# Autodesk Inventor assembly: main assembly
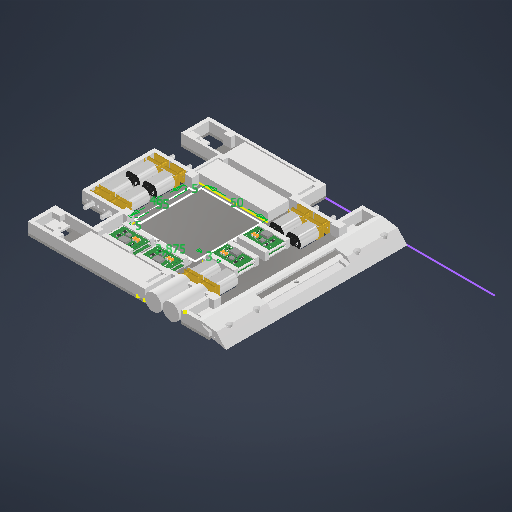
[picture p0: Inventor's stored thumbnail of the model, 512x512]
Saved by Autodesk Inventor 2026.2 (Build 302298010, 298A)
## iProperties
Created: 2026-04-27
Part Number: main assembly
Document SubType Name: Assembly
Designer: karol
Author: karol
## Documents named in this file (21)
- C:\Users\karol\OneDrive\Dokumenty\GitHub\bolt\bolt\cad\assembly\main assembly.iam
- C:\Users\karol\OneDrive\Dokumenty\GitHub\bolt\bolt\cad\ready parts\base.ipt
- C:\Users\karol\OneDrive\Dokumenty\GitHub\bolt\bolt\cad\ready parts\lewasciana.ipt
- C:\Users\karol\OneDrive\Dokumenty\GitHub\bolt\bolt\cad\ready parts\prawasciana.ipt
- C:\Users\karol\OneDrive\Dokumenty\GitHub\bolt\bolt\cad\ready parts\rmwall.ipt
- C:\Users\karol\OneDrive\Dokumenty\GitHub\bolt\bolt\cad\ready parts\lmwall.ipt
- C:\Users\karol\OneDrive\Dokumenty\GitHub\bolt\bolt\cad\ready parts\Pololu #2218 Micro Metal Gearmotor HP.ipt
- C:\Users\karol\OneDrive\Dokumenty\GitHub\bolt\bolt\cad\assembly\backmotors.iam
- C:\Users\karol\OneDrive\Dokumenty\GitHub\bolt\bolt\cad\ready parts\lewascianakoło.ipt
- C:\Users\karol\OneDrive\Dokumenty\GitHub\bolt\bolt\cad\ready parts\prawascianakolo.ipt
- C:\Users\karol\OneDrive\Dokumenty\GitHub\bolt\bolt\cad\ready parts\lfmw.ipt
- C:\Users\karol\OneDrive\Dokumenty\GitHub\bolt\bolt\cad\ready parts\rfmw.ipt
- C:\Users\karol\OneDrive\Dokumenty\GitHub\bolt\bolt\cad\ready parts\lipo.ipt
- C:\Users\karol\OneDrive\Dokumenty\GitHub\bolt\bolt\cad\assembly\plugassmbly.iam
- C:\Users\karol\OneDrive\Dokumenty\GitHub\bolt\bolt\cad\assembly\drvassembly.iam
- C:\Users\karol\OneDrive\Dokumenty\GitHub\bolt\bolt\cad\printing parts\rim-v1.ipt
- C:\Users\karol\OneDrive\Dokumenty\GitHub\bolt\bolt\cad\assembly\drvassemblylf.iam
- drvassemblylf.iam
- C:\Users\karol\OneDrive\Dokumenty\GitHub\bolt\bolt\cad\assembly\drvassemblyrf.iam
- drvassemblyrf.iam
- C:\Users\karol\OneDrive\Dokumenty\GitHub\bolt\bolt\cad\ready parts\zawiasv2.ipt
## Components (25 placed, 18 different names)
1. base:1 — Mate:1, Mate:2, Mate:3, Mate:4, Mate:5, Mate:7, Mate:15, Mate:16, Mate:17, Mate:18, Mate:21, Mate:22, Mate:23, Mate:24, Mate:28, Mate:29, Mate:30, Mate:32, Mate:33, Mate:34, Mate:35, Mate:36, Mate:37, Mate:38, Mate:39, Mate:40, Mate:41, Mate:45, Mate:47, Mate:48, Mate:68, Mate:73, Mate:74, Mate:75, Mate:80, Mate:81, Mate:82, Mate:83
2. lewasciana:1 — Mate:1, Mate:2, Mate:46, Mate:54, Mate:55, Mate:70, Mate:71, Mate:72
3. prawasciana:1 — Mate:3, Mate:4, Mate:49, Mate:56
4. rmwall:1 — Mate:5, Mate:48, Mate:49, Mate:50, Mate:51, Mate:79
5. lmwall:1 — Mate:7, Mate:52, Mate:53, Mate:54, Mate:55, Flush:1, Flush:2, Mate:61, Mate:76
6. Pololu #2218 Micro Metal Gearmotor HP:3 — Mate:17, Mate:18
7. Pololu #2218 Micro Metal Gearmotor HP:4 — Mate:15, Mate:16
8. Pololu #2218 Micro Metal Gearmotor HP:7 — Mate:21, Mate:22
9. Pololu #2218 Micro Metal Gearmotor HP:8 — Mate:23, Mate:24, Mate:60, Angle:1
10. lewascianakoło:1 — Mate:32, Mate:33, Mate:69
11. prawascianakolo:1 — Mate:28, Mate:29, Mate:30, Mate:42, Mate:43
12. backmotors:1 [sub-assembly] — Mate:34, Mate:35
13. lfmw:1 — Mate:36, Mate:37, Mate:38, Mate:52, Mate:53, Mate:77
14. rfmw:1 — Mate:39, Mate:40, Mate:41, Mate:50, Mate:51, Mate:78
15. lipo:2 — Mate:46, Mate:47
16. lipo:3 — Mate:42, Mate:43
17. lipo:4 — Mate:45, Mate:56
18. plugassmbly:1 [sub-assembly] — Mate:84, Mate:85, Mate:86, Mate:87
19. drvassembly:1 [sub-assembly] — Mate:68, Mate:69, Mate:70
20. drvassembly:2 [sub-assembly] — Mate:71, Mate:72, Mate:73
21. rim-v1:1 — Flush:1, Flush:2
22. rim-v1:2 — Mate:60, Angle:1, Mate:61
23. drvassemblylf:1 [sub-assembly] — Mate:75, Mate:78, Mate:79
24. drvassemblyrf:3 [sub-assembly] — Mate:74, Mate:76, Mate:77
25. zawiasv2:1 — Mate:80, Mate:81, Mate:82, Mate:83, Mate:84, Mate:85, Mate:86, Mate:87
## Relationships (66: Mate 63, Flush 2, Angle 1)
- Mate:1: base:1 ↔ lewasciana:1
- Mate:2: base:1 ↔ lewasciana:1
- Mate:3: base:1 ↔ prawasciana:1
- Mate:4: base:1 ↔ prawasciana:1
- Mate:5: base:1 ↔ rmwall:1
- Mate:7: base:1 ↔ lmwall:1
- Mate:15: base:1 ↔ Pololu #2218 Micro Metal Gearmotor HP:4
- Mate:16: base:1 ↔ Pololu #2218 Micro Metal Gearmotor HP:4
- Mate:17: base:1 ↔ Pololu #2218 Micro Metal Gearmotor HP:3
- Mate:18: base:1 ↔ Pololu #2218 Micro Metal Gearmotor HP:3
- Mate:21: base:1 ↔ Pololu #2218 Micro Metal Gearmotor HP:7
- Mate:22: base:1 ↔ Pololu #2218 Micro Metal Gearmotor HP:7
- Mate:23: base:1 ↔ Pololu #2218 Micro Metal Gearmotor HP:8
- Mate:24: base:1 ↔ Pololu #2218 Micro Metal Gearmotor HP:8
- Mate:28: base:1 ↔ prawascianakolo:1
- Mate:29: base:1 ↔ prawascianakolo:1
- Mate:30: base:1 ↔ prawascianakolo:1
- Mate:32: base:1 ↔ lewascianakoło:1
- Mate:33: base:1 ↔ lewascianakoło:1
- Mate:34: base:1 ↔ backmotors:1
- Mate:35: base:1 ↔ backmotors:1
- Mate:36: base:1 ↔ lfmw:1
- Mate:37: base:1 ↔ lfmw:1
- Mate:38: base:1 ↔ lfmw:1
- Mate:39: base:1 ↔ rfmw:1
- Mate:40: base:1 ↔ rfmw:1
- Mate:41: base:1 ↔ rfmw:1
- Mate:42: prawascianakolo:1 ↔ lipo:3
- Mate:43: prawascianakolo:1 ↔ lipo:3
- Mate:45: base:1 ↔ lipo:4
- Mate:46: lewasciana:1 ↔ lipo:2
- Mate:47: base:1 ↔ lipo:2
- Mate:48: base:1 ↔ rmwall:1
- Mate:49: prawasciana:1 ↔ rmwall:1
- Mate:50: rmwall:1 ↔ rfmw:1
- Mate:51: rmwall:1 ↔ rfmw:1
- Mate:52: lmwall:1 ↔ lfmw:1
- Mate:53: lmwall:1 ↔ lfmw:1
- Mate:54: lewasciana:1 ↔ lmwall:1
- Mate:55: lewasciana:1 ↔ lmwall:1
- Mate:56: prawasciana:1 ↔ lipo:4
- Flush:1: lmwall:1 ↔ rim-v1:1
- Flush:2 (0.5 mm): lmwall:1 ↔ rim-v1:1
- Mate:60: Pololu #2218 Micro Metal Gearmotor HP:8 ↔ rim-v1:2
- Angle:1 (180 deg): Pololu #2218 Micro Metal Gearmotor HP:8 ↔ rim-v1:2
- Mate:61: lmwall:1 ↔ rim-v1:2
- Mate:68: base:1 ↔ drvassembly:1
- Mate:69 (5 mm): lewascianakoło:1 ↔ drvassembly:1
- Mate:70 (20 mm): lewasciana:1 ↔ drvassembly:1
- Mate:71 (4 mm): lewasciana:1 ↔ drvassembly:2
- Mate:72 (20 mm): lewasciana:1 ↔ drvassembly:2
- Mate:73: base:1 ↔ drvassembly:2
- Mate:74: base:1 ↔ drvassemblyrf:3
- Mate:75: base:1 ↔ drvassemblylf:1
- Mate:76 (27 mm): lmwall:1 ↔ drvassemblyrf:3
- Mate:77 (8 mm): lfmw:1 ↔ drvassemblyrf:3
- Mate:78 (8 mm): rfmw:1 ↔ drvassemblylf:1
- Mate:79 (27 mm): rmwall:1 ↔ drvassemblylf:1
- Mate:80: base:1 ↔ zawiasv2:1
- Mate:81: base:1 ↔ zawiasv2:1
- Mate:82: base:1 ↔ zawiasv2:1
- Mate:83: base:1 ↔ zawiasv2:1
- Mate:84: plugassmbly:1 ↔ zawiasv2:1
- Mate:85: plugassmbly:1 ↔ zawiasv2:1
- Mate:86: plugassmbly:1 ↔ zawiasv2:1
- Mate:87: plugassmbly:1 ↔ zawiasv2:1
